# Autodesk Inventor assembly: XYZ_Draft1
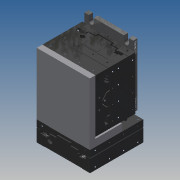
[picture p0: Inventor's stored thumbnail of the model, 180x180]
Saved by Autodesk Inventor 2019 (Build 230136000, 136)
## iProperties
Created: 2019-12-19
Part Number: XYZ_Draft1
Document SubType Name: Assembly
Designer: voigt
Author: voigt
## Documents named in this file (4)
- J:\Microscope_Design\CAD_Files\mesoSPIM_design_benchtop_V1\library\Thorlabs\motorized_stages\XYZ_Draft1.iam
- J:\Microscope_Design\CAD_Files\mesoSPIM_design_benchtop_V1\library\Thorlabs\motorized_stages\ZFM2020-Stage.ipt
- J:\Microscope_Design\CAD_Files\mesoSPIM_design_benchtop_V1\library\Thorlabs\motorized_stages\135962 - Table Adapter Plate PRM1-Z7.ipt
- J:\Microscope_Design\CAD_Files\mesoSPIM_design_benchtop_V1\library\Thorlabs\motorized_stages\MountingBracket.ipt
## Components (5 placed, 3 different names)
1. ZFM2020-Stage:1 — Mate:1, Flush:1, Flush:6, Mate:4
2. ZFM2020-Stage:2 — Mate:1, Flush:1, Flush:2, Flush:3, Mate:2, Mate:6, Flush:8, Flush:9
3. ZFM2020-Stage:3 — Flush:2, Flush:3, Mate:2, Mate:5, Flush:7
4. 135962 - Table Adapter Plate PRM1-Z7:1 — Mate:6, Flush:8, Flush:9
5. MountingBracket:1 — Flush:6, Mate:4, Mate:5, Flush:7
## Relationships (12: Flush 7, Mate 5)
- Mate:1 (13 mm): ZFM2020-Stage:1 ↔ ZFM2020-Stage:2
- Flush:1: ZFM2020-Stage:1 ↔ ZFM2020-Stage:2
- Flush:2: ZFM2020-Stage:2 ↔ ZFM2020-Stage:3
- Flush:3: ZFM2020-Stage:2 ↔ ZFM2020-Stage:3
- Mate:2: ZFM2020-Stage:2 ↔ ZFM2020-Stage:3
- Flush:6: ZFM2020-Stage:1 ↔ MountingBracket:1
- Mate:4: ZFM2020-Stage:1 ↔ MountingBracket:1
- Mate:5: ZFM2020-Stage:3 ↔ MountingBracket:1
- Flush:7: ZFM2020-Stage:3 ↔ MountingBracket:1
- Mate:6: ZFM2020-Stage:2 ↔ 135962 - Table Adapter Plate PRM1-Z7:1
- Flush:8: ZFM2020-Stage:2 ↔ 135962 - Table Adapter Plate PRM1-Z7:1
- Flush:9 (3 mm): ZFM2020-Stage:2 ↔ 135962 - Table Adapter Plate PRM1-Z7:1
